# Autodesk Inventor assembly: Robot
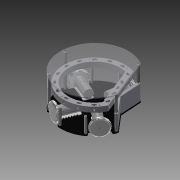
[picture p0: Inventor's stored thumbnail of the model, 180x180]
Saved by Autodesk Inventor 2015 (Build 190159000, 159)
## iProperties
Created: 2016-08-02
Part Number: Robot
Document SubType Name: Assembly
Designer: James Yelland
Author: James Yelland
## Documents named in this file (11)
- C:\Users\James Yelland\git\Layers-2017\Models\Robot.iam
- C:\Users\James Yelland\git\Layers-2017\Models\Bottom Plate.ipt
- C:\Users\James Yelland\git\Layers-2017\Models\Standoff 45.ipt
- C:\Users\James Yelland\git\Layers-2017\Models\Front Support.ipt
- C:\Users\James Yelland\git\Layers-2017\Models\Motor Mount Bracket.ipt
- C:\Users\James Yelland\git\Layers-2017\Models\Motor.ipt
- C:\Users\James Yelland\git\Layers-2017\Models\Wheel.ipt
- C:\Users\James Yelland\git\Layers-2017\Models\Middle Plate.ipt
- C:\Users\James Yelland\git\Layers-2017\Models\TSOP Ring.ipt
- C:\Users\James Yelland\git\Layers-2017\Models\Top Plate.ipt
- C:\Users\James Yelland\git\Layers-2017\Models\Standoff 93.ipt
## Components (25 placed, 10 different names)
1. Bottom Plate:1 — Mate:1, Mate:2, Mate:3, Mate:4, Mate:5, Mate:6, Mate:7, Mate:8, Mate:9, Mate:10, Mate:11, Mate:26, Mate:27, Mate:28, Mate:29, Mate:30, Mate:31, Mate:32, Mate:33, Mate:34, Mate:35, Mate:36, Mate:37, Mate:71, Mate:72, Mate:73, Mate:74
2. Standoff 45:1 — Mate:2, Mate:7
3. Standoff 45:2 — Mate:1, Mate:5
4. Standoff 45:3 — Mate:3, Mate:6
5. Standoff 45:4 — Mate:4, Mate:8
6. Front Support:1 — Mate:9, Mate:10, Mate:11, Mate:58, Mate:59, Mate:60
7. Motor Mount Bracket:1 — Mate:26, Mate:30, Mate:31, Mate:39, Mate:44, Mate:45
8. Motor Mount Bracket:2 — Mate:27, Mate:36, Mate:37, Mate:38, Mate:46, Mate:47
9. Motor Mount Bracket:3 — Mate:28, Mate:34, Mate:35, Mate:40, Mate:48, Mate:49
10. Motor Mount Bracket:4 — Mate:29, Mate:32, Mate:33, Mate:41, Mate:42, Mate:43
11. Motor:1 — Mate:38, Mate:46, Mate:47, Flush:2, Mate:55
12. Motor:2 — Mate:40, Mate:48, Mate:49, Flush:1, Mate:54
13. Motor:3 — Mate:41, Mate:42, Mate:43, Mate:56, Flush:3
14. Motor:4 — Mate:39, Mate:44, Mate:45, Mate:57, Flush:4
15. Wheel:1 — Flush:1, Mate:54
16. Wheel:2 — Flush:2, Mate:55
17. Wheel:3 — Mate:56, Flush:3
18. Wheel:4 — Mate:57, Flush:4
19. Middle Plate:1 — Mate:58, Mate:59, Mate:60, Mate:61, Mate:62, Mate:63, Mate:64, Mate:65, Mate:66, Mate:67
20. TSOP Ring:1 — Mate:61, Mate:62, Mate:63
21. Standoff 45:7 — Mate:64, Mate:65, Mate:68, Mate:69
22. Standoff 45:8 — Mate:66, Mate:67, Mate:70
23. Top Plate:1 — Mate:68, Mate:69, Mate:70
24. Standoff 93:1 — Mate:71, Mate:73
25. Standoff 93:2 — Mate:72, Mate:74
## Relationships (60: Mate 56, Flush 4)
- Mate:1: Bottom Plate:1 ↔ Standoff 45:2
- Mate:2: Bottom Plate:1 ↔ Standoff 45:1
- Mate:3: Bottom Plate:1 ↔ Standoff 45:3
- Mate:4: Bottom Plate:1 ↔ Standoff 45:4
- Mate:5: Bottom Plate:1 ↔ Standoff 45:2
- Mate:6: Bottom Plate:1 ↔ Standoff 45:3
- Mate:7: Bottom Plate:1 ↔ Standoff 45:1
- Mate:8: Bottom Plate:1 ↔ Standoff 45:4
- Mate:9: Bottom Plate:1 ↔ Front Support:1
- Mate:10: Bottom Plate:1 ↔ Front Support:1
- Mate:11: Bottom Plate:1 ↔ Front Support:1
- Mate:26: Bottom Plate:1 ↔ Motor Mount Bracket:1
- Mate:27: Bottom Plate:1 ↔ Motor Mount Bracket:2
- Mate:28: Bottom Plate:1 ↔ Motor Mount Bracket:3
- Mate:29: Bottom Plate:1 ↔ Motor Mount Bracket:4
- Mate:30: Bottom Plate:1 ↔ Motor Mount Bracket:1
- Mate:31: Bottom Plate:1 ↔ Motor Mount Bracket:1
- Mate:32: Bottom Plate:1 ↔ Motor Mount Bracket:4
- Mate:33: Bottom Plate:1 ↔ Motor Mount Bracket:4
- Mate:34: Bottom Plate:1 ↔ Motor Mount Bracket:3
- Mate:35: Bottom Plate:1 ↔ Motor Mount Bracket:3
- Mate:36: Bottom Plate:1 ↔ Motor Mount Bracket:2
- Mate:37: Bottom Plate:1 ↔ Motor Mount Bracket:2
- Mate:38: Motor Mount Bracket:2 ↔ Motor:1
- Mate:39: Motor Mount Bracket:1 ↔ Motor:4
- Mate:40: Motor Mount Bracket:3 ↔ Motor:2
- Mate:41: Motor Mount Bracket:4 ↔ Motor:3
- Mate:42: Motor Mount Bracket:4 ↔ Motor:3
- Mate:43: Motor Mount Bracket:4 ↔ Motor:3
- Mate:44: Motor Mount Bracket:1 ↔ Motor:4
- Mate:45: Motor Mount Bracket:1 ↔ Motor:4
- Mate:46: Motor Mount Bracket:2 ↔ Motor:1
- Mate:47: Motor Mount Bracket:2 ↔ Motor:1
- Mate:48: Motor Mount Bracket:3 ↔ Motor:2
- Mate:49: Motor Mount Bracket:3 ↔ Motor:2
- Flush:1: Motor:2 ↔ Wheel:1
- Mate:54: Motor:2 ↔ Wheel:1
- Flush:2: Motor:1 ↔ Wheel:2
- Mate:55: Motor:1 ↔ Wheel:2
- Mate:56: Motor:3 ↔ Wheel:3
- Flush:3: Motor:3 ↔ Wheel:3
- Mate:57: Motor:4 ↔ Wheel:4
- Flush:4: Motor:4 ↔ Wheel:4
- Mate:58: Front Support:1 ↔ Middle Plate:1
- Mate:59: Front Support:1 ↔ Middle Plate:1
- Mate:60: Front Support:1 ↔ Middle Plate:1
- Mate:61: Middle Plate:1 ↔ TSOP Ring:1
- Mate:62: Middle Plate:1 ↔ TSOP Ring:1
- Mate:63: Middle Plate:1 ↔ TSOP Ring:1
- Mate:64: Middle Plate:1 ↔ Standoff 45:7
- Mate:65: Middle Plate:1 ↔ Standoff 45:7
- Mate:66: Middle Plate:1 ↔ Standoff 45:8
- Mate:67: Middle Plate:1 ↔ Standoff 45:8
- Mate:68: Standoff 45:7 ↔ Top Plate:1
- Mate:69: Standoff 45:7 ↔ Top Plate:1
- Mate:70: Standoff 45:8 ↔ Top Plate:1
- Mate:71: Bottom Plate:1 ↔ Standoff 93:1
- Mate:72: Bottom Plate:1 ↔ Standoff 93:2
- Mate:73: Bottom Plate:1 ↔ Standoff 93:1
- Mate:74: Bottom Plate:1 ↔ Standoff 93:2
